# Autodesk Inventor assembly: Assembly2
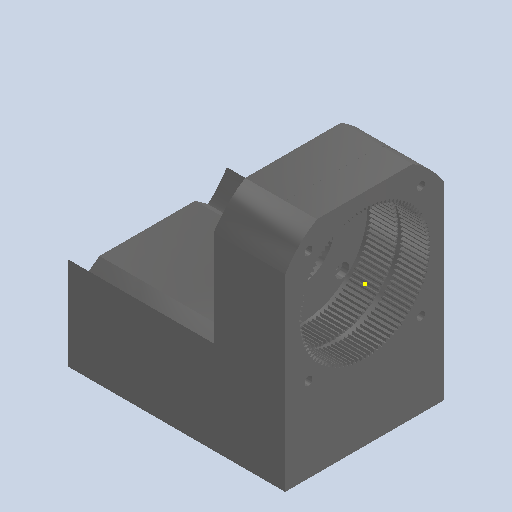
[picture p0: Inventor's stored thumbnail of the model, 512x512]
Saved by Autodesk Inventor 2022 (Build 260153000, 153)
## iProperties
Created: 2022-02-10
Part Number: Assembly2
Document SubType Name: Assembly
Designer: Mlees
Author: Mlees
## Documents named in this file (3)
- C:\Users\Mlees\Desktop\504Engineering\Stepper-Servo_Based_Robotic_Arm\Designs\Version_5\Created_Parts\Assembly2.iam
- C:\Users\Mlees\Desktop\504Engineering\Stepper-Servo_Based_Robotic_Arm\Designs\Version_5\Created_Parts\96Gears_Stage_1_modified.ipt
- C:\Users\Mlees\Desktop\504Engineering\Stepper-Servo_Based_Robotic_Arm\Designs\Version_5\Created_Parts\96Gears_Stage_2_modified.ipt
## Components (2 placed, 2 different names)
1. 96Gears_Stage_1_modified:1 — Rigid:1
2. 96Gears_Stage_2_modified:1 — Rigid:1
## Relationships (1: WeldJoint 1)
- Rigid:1 [WeldJoint]: 96Gears_Stage_1_modified:1 ↔ 96Gears_Stage_2_modified:1
